# Autodesk Inventor assembly: eStopBox
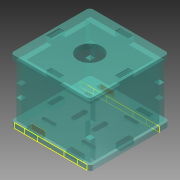
[picture p0: Inventor's stored thumbnail of the model, 180x180]
Saved by Autodesk Inventor 2015 SP1 (Build 190203100, 203)
## iProperties
Created: 2016-04-13
Part Number: eStopBox
Document SubType Name: Assembly
Designer: tuttlem
Author: tuttlem
## Documents named in this file (6)
- C:\Users\tuttlem\Desktop\MotionBase\CAD\eStop\eStopBox.iam
- C:\Users\tuttlem\Desktop\MotionBase\CAD\eStop\bottom.ipt
- C:\Users\tuttlem\Desktop\MotionBase\CAD\eStop\sideL.ipt
- C:\Users\tuttlem\Desktop\MotionBase\CAD\eStop\sideR.ipt
- C:\Users\tuttlem\Desktop\MotionBase\CAD\eStop\back.ipt
- C:\Users\tuttlem\Desktop\MotionBase\CAD\eStop\top.ipt
## Components (6 placed, 5 different names)
1. bottom:1 — Flush:1, Flush:2, Mate:1, Mate:2
2. sideL — Flush:1, Flush:2, Flush:3
3. sideR:1 — Mate:1, Mate:2, Mate:3
4. back:1 — Flush:3
5. back:2
6. top:1 — Mate:3
## Relationships (6: Flush 3, Mate 3)
- Flush:1: bottom:1 ↔ sideL
- Flush:2: bottom:1 ↔ sideL
- Mate:1: bottom:1 ↔ sideR:1
- Mate:2: bottom:1 ↔ sideR:1
- Flush:3: sideL ↔ back:1
- Mate:3: sideR:1 ↔ top:1
